# Autodesk Inventor assembly: PCB
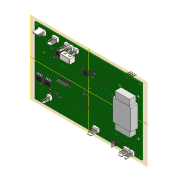
[picture p0: Inventor's stored thumbnail of the model, 180x180]
Saved by Autodesk Inventor 2020 (Build 240168000, 168)
## iProperties
Company: A Company
Created: 2020-04-15
Part Number: PCB
Description: BREEZE CIRCUIT BOARD
Document SubType Name: Assembly
Designer: John K
Authority: Unknown
Sending System: KiCad to STEP converter
Preprocessor: Open CASCADE STEP processor 6.9
Title: ventilator_shield.step
Author: An Author
## Documents named in this file (20)
- C:\GrabCAD\MTL Ventilator Design\BREEZE\Manufactured Parts\PCB\PCB.iam
- C:\GrabCAD\MTL Ventilator Design\BREEZE\Manufactured Parts\PCB\R_0805_2012Metric.iam
- C:\GrabCAD\MTL Ventilator Design\BREEZE\Manufactured Parts\PCB\C_0805_2012Metric.iam
- C:\GrabCAD\MTL Ventilator Design\BREEZE\Manufactured Parts\PCB\PinHeader_1x04_P2.54mm_Vertical.iam
- C:\GrabCAD\MTL Ventilator Design\BREEZE\Manufactured Parts\PCB\SOT-23-5.iam
- C:\GrabCAD\MTL Ventilator Design\BREEZE\Manufactured Parts\PCB\SOT-363_SC-70-6.iam
- C:\GrabCAD\MTL Ventilator Design\BREEZE\Manufactured Parts\PCB\SOT-323_SC-70.iam
- C:\GrabCAD\MTL Ventilator Design\BREEZE\Manufactured Parts\PCB\TSOT-23-5.iam
- C:\GrabCAD\MTL Ventilator Design\BREEZE\Manufactured Parts\PCB\DIP-8_W10.16mm.iam
- C:\GrabCAD\MTL Ventilator Design\BREEZE\Manufactured Parts\PCB\R_Shunt_Ohmite_LVK12.iam
- C:\GrabCAD\MTL Ventilator Design\BREEZE\Manufactured Parts\PCB\TO-252-2.iam
- C:\GrabCAD\MTL Ventilator Design\BREEZE\Manufactured Parts\PCB\Relay_DPDT_Omron_G6S-2F.iam
- C:\GrabCAD\MTL Ventilator Design\BREEZE\Manufactured Parts\PCB\PinHeader_1x03_P2.54mm_Vertical.iam
- C:\GrabCAD\MTL Ventilator Design\BREEZE\Manufactured Parts\PCB\PinHeader_1x06_P2.54mm_Vertical.iam
- C:\GrabCAD\MTL Ventilator Design\BREEZE\Manufactured Parts\PCB\Molex_KK-254_AE-6410-02A_1x02_P2.54mm_Vertical.iam
- C:\GrabCAD\MTL Ventilator Design\BREEZE\Manufactured Parts\PCB\Molex_KK-254_AE-6410-03A_1x03_P2.54mm_Vertical.iam
- C:\GrabCAD\MTL Ventilator Design\BREEZE\Manufactured Parts\PCB\Molex_KK-254_AE-6410-04A_1x04_P2.54mm_Vertical.iam
- C:\GrabCAD\MTL Ventilator Design\BREEZE\Manufactured Parts\PCB\COMPOUND.ipt
- C:\GrabCAD\MTL Ventilator Design\BREEZE\Commercial Parts\Electronics\Arduino\Arduino MEGA2650 v17.iam
- C:\GrabCAD\MTL Ventilator Design\BREEZE\Commercial Parts\Electronics\Motor Controller.ipt
## Components (62 placed, 62 different names)
1. 2 [sub-assembly]
2. 4 [sub-assembly]
3. 5 [sub-assembly]
4. 7 [sub-assembly]
5. 8 [sub-assembly]
6. 10 [sub-assembly]
7. 11 [sub-assembly]
8. 13 [sub-assembly]
9. 14 [sub-assembly]
10. 16 [sub-assembly]
11. 18 [sub-assembly]
12. 19 [sub-assembly]
13. 20 [sub-assembly]
14. 22 [sub-assembly]
15. 23 [sub-assembly]
16. 24 [sub-assembly]
17. 25 [sub-assembly]
18. 26 [sub-assembly]
19. 27 [sub-assembly]
20. 28 [sub-assembly]
21. 29 [sub-assembly]
22. 30 [sub-assembly]
23. 32 [sub-assembly]
24. 33 [sub-assembly]
25. 34 [sub-assembly]
26. 35 [sub-assembly]
27. 36 [sub-assembly]
28. 37 [sub-assembly]
29. 38 [sub-assembly]
30. 39 [sub-assembly]
31. 40 [sub-assembly]
32. 41 [sub-assembly]
33. 42 [sub-assembly]
34. 43 [sub-assembly]
35. 45 [sub-assembly]
36. 46 [sub-assembly]
37. 48 [sub-assembly]
38. 50 [sub-assembly]
39. 51 [sub-assembly]
40. 53 [sub-assembly]
41. 55 [sub-assembly]
42. 57 [sub-assembly]
43. 59 [sub-assembly]
44. 60 [sub-assembly]
45. 61 [sub-assembly]
46. 62 [sub-assembly]
47. 63 [sub-assembly]
48. 64 [sub-assembly]
49. 65 [sub-assembly]
50. 66 [sub-assembly]
51. 67 [sub-assembly]
52. 68 [sub-assembly]
53. 69 [sub-assembly]
54. 70 [sub-assembly]
55. 71 [sub-assembly]
56. 72 [sub-assembly]
57. 73 [sub-assembly]
58. 74 [sub-assembly]
59. 75 [sub-assembly]
60. 83 — Mate:1, Mate:2, Mate:3, Mate:4, Flush:1, Flush:2, Flush:3, Flush:4, Flush:5
61. Arduino MEGA2650 v17:1 [sub-assembly] — Mate:1, Mate:2, Mate:3
62. Motor Controller:1 — Mate:4, Flush:1, Flush:2
## Relationships (9: Flush 5, Mate 4)
- Mate:1 (2.59 mm): 83 ↔ Arduino MEGA2650 v17:1
- Mate:2: 83 ↔ Arduino MEGA2650 v17:1
- Mate:3: 83 ↔ Arduino MEGA2650 v17:1
- Mate:4: 83 ↔ Motor Controller:1
- Flush:1 (5.75 mm): 83 ↔ Motor Controller:1
- Flush:2 (30 mm): 83 ↔ Motor Controller:1
- Flush:3 (-80 mm): 83
- Flush:4 (-50 mm): 83
- Flush:5 (-0.8 mm): 83
